# Autodesk Inventor assembly: GankenKun_ver3_0
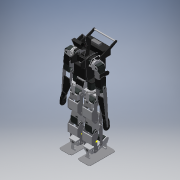
[picture p0: Inventor's stored thumbnail of the model, 180x180]
Saved by Autodesk Inventor 2018 (Build 220112000, 112)
## iProperties
Created: 2018-10-17
Part Number: GankenKun_ver3_0
Material: 一般
Document SubType Name: Assembly
Designer: taka
Author: taka
## Documents named in this file (20)
- C:\Users\taka\Documents\git\OpenPlatform\mechanism\OpenPlatform_ver3_0\SpimplifiedModel\GankenKun_ver3_0.iam
- C:\Users\taka\Documents\git\OpenPlatform\mechanism\OpenPlatform_ver3_0\SpimplifiedModel\上半身\Body.ipt
- C:\Users\taka\Documents\git\OpenPlatform\mechanism\OpenPlatform_ver3_0\SpimplifiedModel\上半身\Head.ipt
- C:\Users\taka\Documents\git\OpenPlatform\mechanism\OpenPlatform_ver3_0\SpimplifiedModel\上半身\Shoulder.ipt
- C:\Users\taka\Documents\git\OpenPlatform\mechanism\OpenPlatform_ver3_0\SpimplifiedModel\上半身\UpperArm.ipt
- C:\Users\taka\Documents\git\OpenPlatform\mechanism\OpenPlatform_ver3_0\SpimplifiedModel\上半身\ForeArm.ipt
- C:\Users\taka\Documents\git\OpenPlatform\mechanism\OpenPlatform_ver3_0\SpimplifiedModel\下半身\KneeR.ipt
- C:\Users\taka\Documents\git\OpenPlatform\mechanism\OpenPlatform_ver3_0\SpimplifiedModel\下半身\AnkleL.ipt
- C:\Users\taka\Documents\git\OpenPlatform\mechanism\OpenPlatform_ver3_0\SpimplifiedModel\下半身\AnkleR.ipt
- C:\Users\taka\Documents\git\OpenPlatform\mechanism\OpenPlatform_ver3_0\SpimplifiedModel\下半身\FootL.ipt
- C:\Users\taka\Documents\git\OpenPlatform\mechanism\OpenPlatform_ver3_0\SpimplifiedModel\下半身\FootR.ipt
- C:\Users\taka\Documents\git\OpenPlatform\mechanism\OpenPlatform_ver3_0\SpimplifiedModel\下半身\Hip_Y.ipt
- C:\Users\taka\Documents\git\OpenPlatform\mechanism\OpenPlatform_ver3_0\SpimplifiedModel\下半身\KneeL.ipt
- C:\Users\taka\Documents\git\OpenPlatform\mechanism\OpenPlatform_ver3_0\SpimplifiedModel\下半身\Thigh_Rear.ipt
- C:\Users\taka\Documents\git\OpenPlatform\mechanism\OpenPlatform_ver3_0\SpimplifiedModel\下半身\Shin_Fore.ipt
- C:\Users\taka\Documents\git\OpenPlatform\mechanism\OpenPlatform_ver3_0\SpimplifiedModel\下半身\Shin_Rear.ipt
- C:\Users\taka\Documents\git\OpenPlatform\mechanism\OpenPlatform_ver3_0\SpimplifiedModel\下半身\Tarsus.ipt
- C:\Users\taka\Documents\git\OpenPlatform\mechanism\OpenPlatform_ver3_0\SpimplifiedModel\下半身\Thigh_Fore.ipt
- C:\Users\taka\Documents\git\OpenPlatform\mechanism\OpenPlatform_ver3_0\SpimplifiedModel\下半身\HipL_L.ipt
- C:\Users\taka\Documents\git\OpenPlatform\mechanism\OpenPlatform_ver3_0\SpimplifiedModel\下半身\HipR_R.ipt
## Components (28 placed, 19 different names)
1. Body:1 — 挿入:1, 角度:1, 挿入:2, 角度:3, 挿入:4, 角度:5, 挿入:8, 角度:8, 挿入:20, 角度:12, 角度:22, 角度:23, 角度:28, 角度:29
2. Head:1 — 挿入:1, 角度:1
3. Shoulder:1 — 挿入:4, 挿入:5, 角度:22
4. UpperArm:1 — 挿入:5, 角度:5, 挿入:6, 角度:7
5. ForeArm:1 — 挿入:6, 角度:7
6. Shoulder:2 — 挿入:2, 挿入:3, 角度:23
7. ForeArm:2 — 挿入:7, 角度:6
8. UpperArm:2 — 挿入:3, 角度:3, 挿入:7, 角度:6
9. KneeR:1 — 挿入:28, 挿入:29, 挿入:31, 挿入:41, 角度:26, 角度:30, 角度:33
10. AnkleL:1 — 挿入:24, 挿入:37, 角度:19, 角度:32
11. AnkleR:1 — 挿入:36, 挿入:38, 角度:18, 角度:33
12. FootL:1 — 挿入:37, 角度:19
13. FootR:1 — 挿入:38, 角度:18
14. Hip_Y:1 — 挿入:8, 角度:8, 挿入:40
15. KneeL:1 — 挿入:12, 挿入:13, 挿入:14, 挿入:15, 角度:27, 角度:31, 角度:32
16. Thigh_Rear:1 — 挿入:13, 挿入:23
17. Shin_Fore:1 — 挿入:14, 挿入:17, 角度:31
18. Shin_Rear:1 — 挿入:15, 挿入:16
19. Tarsus:1 — 挿入:16, 挿入:17, 挿入:24
20. Thigh_Fore:1 — 挿入:12, 挿入:22, 角度:25
21. Tarsus:4 — 挿入:34, 挿入:36, 挿入:42
22. Thigh_Rear:2 — 挿入:27, 挿入:29
23. Shin_Rear:2 — 挿入:31, 挿入:34
24. Hip_Y:2 — 挿入:20, 角度:12, 挿入:39
25. Thigh_Fore:2 — 挿入:26, 挿入:28, 角度:24
26. HipL_L:1 — 挿入:22, 挿入:23, 挿入:40, 角度:25, 角度:27, 角度:28
27. HipR_R:1 — 挿入:26, 挿入:27, 挿入:39, 角度:24, 角度:26, 角度:29
28. Shin_Fore:2 — 挿入:41, 挿入:42, 角度:30
## Relationships (52: Insert 31, Angle 21)
- 挿入:1 [Insert]: Body:1 ↔ Head:1
- 角度:1 [Angle] (0 deg): Body:1 ↔ Head:1
- 挿入:2 [Insert]: Body:1 ↔ Shoulder:2
- 挿入:3 [Insert]: Shoulder:2 ↔ UpperArm:2
- 角度:3 [Angle] (85 deg): Body:1 ↔ UpperArm:2
- 挿入:4 [Insert]: Body:1 ↔ Shoulder:1
- 挿入:5 [Insert]: Shoulder:1 ↔ UpperArm:1
- 角度:5 [Angle] (-85 deg): Body:1 ↔ UpperArm:1
- 挿入:6 [Insert]: UpperArm:1 ↔ ForeArm:1
- 挿入:7 [Insert]: ForeArm:2 ↔ UpperArm:2
- 角度:6 [Angle] (180 deg): ForeArm:2 ↔ UpperArm:2
- 角度:7 [Angle] (0 deg): UpperArm:1 ↔ ForeArm:1
- 挿入:8 [Insert]: Body:1 ↔ Hip_Y:1
- 角度:8 [Angle] (0 deg): Body:1 ↔ Hip_Y:1
- 挿入:12 [Insert]: KneeL:1 ↔ Thigh_Fore:1
- 挿入:13 [Insert]: KneeL:1 ↔ Thigh_Rear:1
- 挿入:14 [Insert] (4 mm): KneeL:1 ↔ Shin_Fore:1
- 挿入:15 [Insert]: KneeL:1 ↔ Shin_Rear:1
- 挿入:16 [Insert]: Shin_Rear:1 ↔ Tarsus:1
- 挿入:17 [Insert]: Shin_Fore:1 ↔ Tarsus:1
- 挿入:20 [Insert]: Body:1 ↔ Hip_Y:2
- 角度:12 [Angle] (0 deg): Body:1 ↔ Hip_Y:2
- 挿入:22 [Insert] (4 mm): Thigh_Fore:1 ↔ HipL_L:1
- 挿入:23 [Insert]: Thigh_Rear:1 ↔ HipL_L:1
- 挿入:24 [Insert]: AnkleL:1 ↔ Tarsus:1
- 挿入:26 [Insert] (4 mm): Thigh_Fore:2 ↔ HipR_R:1
- 挿入:27 [Insert]: Thigh_Rear:2 ↔ HipR_R:1
- 挿入:28 [Insert]: KneeR:1 ↔ Thigh_Fore:2
- 挿入:29 [Insert]: KneeR:1 ↔ Thigh_Rear:2
- 挿入:31 [Insert]: KneeR:1 ↔ Shin_Rear:2
- 挿入:34 [Insert]: Tarsus:4 ↔ Shin_Rear:2
- 挿入:36 [Insert]: AnkleR:1 ↔ Tarsus:4
- 挿入:37 [Insert]: AnkleL:1 ↔ FootL:1
- 挿入:38 [Insert]: AnkleR:1 ↔ FootR:1
- 角度:18 [Angle] (0 deg): AnkleR:1 ↔ FootR:1
- 角度:19 [Angle] (0 deg): AnkleL:1 ↔ FootL:1
- 角度:22 [Angle] (0 deg): Body:1 ↔ Shoulder:1
- 角度:23 [Angle] (0 deg): Body:1 ↔ Shoulder:2
- 挿入:39 [Insert]: Hip_Y:2 ↔ HipR_R:1
- 挿入:40 [Insert]: Hip_Y:1 ↔ HipL_L:1
- 挿入:41 [Insert] (4 mm): KneeR:1 ↔ Shin_Fore:2
- 挿入:42 [Insert]: Tarsus:4 ↔ Shin_Fore:2
- 角度:24 [Angle] (0 deg): Thigh_Fore:2 ↔ HipR_R:1
- 角度:25 [Angle] (0 deg): Thigh_Fore:1 ↔ HipL_L:1
- 角度:26 [Angle] (0 deg): KneeR:1 ↔ HipR_R:1
- 角度:27 [Angle] (0 deg): KneeL:1 ↔ HipL_L:1
- 角度:28 [Angle] (0 deg): Body:1 ↔ HipL_L:1
- 角度:29 [Angle] (0 deg): Body:1 ↔ HipR_R:1
- 角度:30 [Angle] (0 deg): KneeR:1 ↔ Shin_Fore:2
- 角度:31 [Angle] (0 deg): KneeL:1 ↔ Shin_Fore:1
- 角度:32 [Angle] (0 deg): AnkleL:1 ↔ KneeL:1
- 角度:33 [Angle] (0 deg): KneeR:1 ↔ AnkleR:1
